# Autodesk Inventor assembly: Bracket Assembly MK29
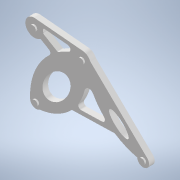
[picture p0: Inventor's stored thumbnail of the model, 180x180]
Saved by Autodesk Inventor 2021 (Build 250183000, 183)
## iProperties
Created: 2021-05-20
Part Number: Bracket Assembly MK29
Document SubType Name: Assembly
Designer: jtri402
Author: jtri402
## Documents named in this file (3)
- C:\Users\Jawal\Documents\UNI\PART III\Semester 1\MECHENG 334\Project B\Concept Design\Bracket Assembly MK29.iam
- C:\Users\Jawal\Documents\UNI\PART III\Semester 1\MECHENG 334\Project B\Concept Design\Pins.ipt
- C:\Users\Jawal\Documents\UNI\PART III\Semester 1\MECHENG 334\Project B\Concept Design\Bracket Design MK29.ipt
## Components (5 placed, 2 different names)
1. Pins:1 — Rigid:2
2. Pins:2 — Rigid:1
3. Pins:3 — Rigid:3
4. Pins:4 — Rigid:4
5. Bracket Design MK29:1 — Rigid:1, Rigid:2, Rigid:3, Rigid:4
## Relationships (4: WeldJoint 4)
- Rigid:1 [WeldJoint]: Pins:2 ↔ Bracket Design MK29:1
- Rigid:2 [WeldJoint]: Pins:1 ↔ Bracket Design MK29:1
- Rigid:3 [WeldJoint]: Pins:3 ↔ Bracket Design MK29:1
- Rigid:4 [WeldJoint]: Pins:4 ↔ Bracket Design MK29:1
